# Autodesk Inventor assembly: s-assy-link3+4+5+gripper
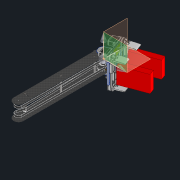
[picture p0: Inventor's stored thumbnail of the model, 180x180]
Saved by Autodesk Inventor 2021 (Build 250183000, 183)
## iProperties
Created: 2021-08-13
Part Number: s-assy-link3+4+5+gripper
Document SubType Name: Assembly
Designer: yuta0
Mass: 1390.53 g
Surface Area: 5373.96 cm^2
Volume: 1228.57 cm^3
Density: 1.13182 g/cm^3
Author: yuta0
## Documents named in this file (3)
- C:\Users\yuta0\Documents\GitHub\catchrobo_hardware\assy-robot\s-assy-link3+4+5+gripper.iam
- C:\Users\yuta0\Documents\GitHub\catchrobo_hardware\assy-robot\s-assy-link3.iam
- C:\Users\yuta0\Documents\GitHub\catchrobo_hardware\assy-robot\s-assy-link4+5+gripper.iam
## Components (2 placed, 2 different names)
1. s-assy-link3:1 [sub-assembly] — メイト:1, メイト:2
2. s-assy-link4+5+gripper:1 [sub-assembly] — メイト:1, メイト:2, 角度:4
## Relationships (3: Mate 2, Angle 1)
- メイト:1 [Mate]: s-assy-link3:1 ↔ s-assy-link4+5+gripper:1
- メイト:2 [Mate]: s-assy-link3:1 ↔ s-assy-link4+5+gripper:1
- 角度:4 [Angle] (110 deg): s-assy-link4+5+gripper:1
